# Autodesk Inventor assembly: window
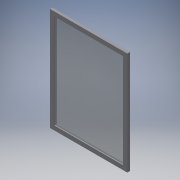
[picture p0: Inventor's stored thumbnail of the model, 180x180]
Saved by Autodesk Inventor 2017 (Build 210142000, 142)
## iProperties
Created: 2019-05-07
Part Number: window
Document SubType Name: Assembly
Designer: Roman
Author: Roman
## Documents named in this file (5)
- C:\Users\Roman\Documents\CAD\tegu rev2\upper walls\window wall\window\window.iam
- C:\Users\Roman\Documents\CAD\tegu rev2\upper walls\window wall\window\window frame tall.ipt
- C:\Users\Roman\Documents\CAD\tegu rev2\upper walls\window wall\window\window frame short.ipt
- C:\Users\Roman\Documents\CAD\tegu rev2\upper walls\window wall\window\window frame corner.ipt
- C:\Users\Roman\Documents\CAD\tegu rev2\upper walls\window wall\window\window glass.ipt
## Components (9 placed, 4 different names)
1. window frame tall:1 — Mate:5, Flush:9, Flush:10
2. window frame tall:2 — Mate:6, Flush:11, Flush:12, Mate:7, Flush:13, Flush:14, Mate:9
3. window frame short:1 — Mate:1, Flush:1, Flush:2, Mate:2, Flush:3, Flush:4
4. window frame short:2 — Mate:3, Flush:5, Flush:6, Mate:4, Flush:7, Flush:8, Mate:8, Mate:10
5. window frame corner:1 — Mate:3, Flush:5, Flush:6
6. window frame corner:2 — Mate:1, Flush:1, Flush:2, Mate:5, Flush:9, Flush:10
7. window frame corner:3 — Mate:2, Flush:3, Flush:4, Mate:6, Flush:11, Flush:12
8. window frame corner:4 — Mate:4, Flush:7, Flush:8, Mate:7, Flush:13, Flush:14
9. window glass:1 — Mate:8, Mate:9, Mate:10
## Relationships (24: Flush 14, Mate 10)
- Mate:1: window frame short:1 ↔ window frame corner:2
- Flush:1: window frame short:1 ↔ window frame corner:2
- Flush:2: window frame short:1 ↔ window frame corner:2
- Mate:2: window frame short:1 ↔ window frame corner:3
- Flush:3: window frame short:1 ↔ window frame corner:3
- Flush:4: window frame short:1 ↔ window frame corner:3
- Mate:3: window frame short:2 ↔ window frame corner:1
- Flush:5: window frame short:2 ↔ window frame corner:1
- Flush:6: window frame short:2 ↔ window frame corner:1
- Mate:4: window frame short:2 ↔ window frame corner:4
- Flush:7: window frame short:2 ↔ window frame corner:4
- Flush:8: window frame short:2 ↔ window frame corner:4
- Mate:5: window frame tall:1 ↔ window frame corner:2
- Flush:9: window frame tall:1 ↔ window frame corner:2
- Flush:10: window frame tall:1 ↔ window frame corner:2
- Mate:6: window frame tall:2 ↔ window frame corner:3
- Flush:11: window frame tall:2 ↔ window frame corner:3
- Flush:12: window frame tall:2 ↔ window frame corner:3
- Mate:7: window frame tall:2 ↔ window frame corner:4
- Flush:13: window frame tall:2 ↔ window frame corner:4
- Flush:14: window frame tall:2 ↔ window frame corner:4
- Mate:8: window frame short:2 ↔ window glass:1
- Mate:9: window frame tall:2 ↔ window glass:1
- Mate:10: window frame short:2 ↔ window glass:1
